# Autodesk Inventor assembly: socket
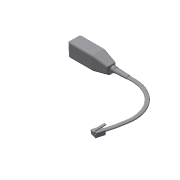
[picture p0: Inventor's stored thumbnail of the model, 180x180]
Saved by Autodesk Inventor 2022 (Build 260148000, 148)
## iProperties
Created: 2005-04-19
Part Number: socket
Document SubType Name: Assembly
Designer: skovacevic
Manufacturer: Standard
Standards Organization: Custom
Author: skovacevic
## Documents named in this file (6)
- C:\Autodesk Inventor 2022 Advanced Assembly Modeling Practice Files\Mirror Assembly Components\socket.iam
- C:\Autodesk Inventor 2022 Advanced Assembly Modeling Practice Files\Mirror Assembly Components\encbase.ipt
- C:\Autodesk Inventor 2022 Advanced Assembly Modeling Practice Files\Mirror Assembly Components\pcb.ipt
- C:\Autodesk Inventor 2022 Advanced Assembly Modeling Practice Files\Mirror Assembly Components\connect.ipt
- C:\Autodesk Inventor 2022 Advanced Assembly Modeling Practice Files\Mirror Assembly Components\wire.ipt
- C:\Autodesk Inventor 2022 Advanced Assembly Modeling Practice Files\Mirror Assembly Components\enctop.ipt
## Components (5 placed, 5 different names)
1. encbase:1 — Insert:1, Angle:1, Insert:3, Mate:1, Flush:1, Flush:2, Mate:2
2. pcb:1 — Insert:1, Angle:1, Angle:2, Insert:2
3. connect:1 — Angle:2, Insert:2
4. wire:1 — Insert:3, Mate:1
5. enctop:1 — Flush:1, Flush:2, Mate:2
## Relationships (9: Insert 3, Angle 2, Mate 2, Flush 2)
- Insert:1 (-6.985 mm): encbase:1 ↔ pcb:1
- Angle:1 (180 deg): encbase:1 ↔ pcb:1
- Angle:2 (0 deg): pcb:1 ↔ connect:1
- Insert:2: pcb:1 ↔ connect:1
- Insert:3: encbase:1 ↔ wire:1
- Mate:1: encbase:1 ↔ wire:1
- Flush:1: encbase:1 ↔ enctop:1
- Flush:2: encbase:1 ↔ enctop:1
- Mate:2: encbase:1 ↔ enctop:1
